# Autodesk Inventor assembly: dish_print
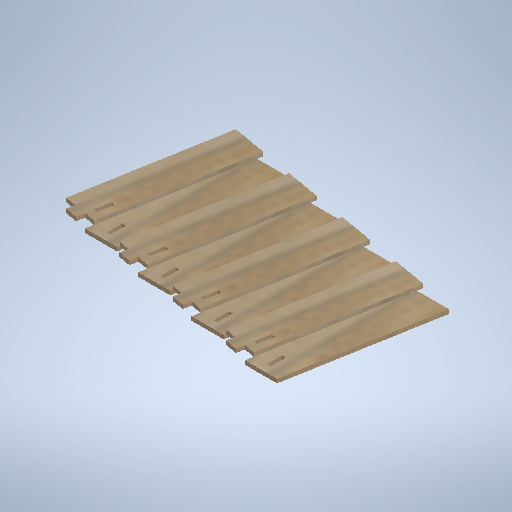
[picture p0: Inventor's stored thumbnail of the model, 512x512]
Saved by Autodesk Inventor 2026.1 (Build 301233020, 233B)
## iProperties
Created: 2025-10-27
Part Number: dish_print
Document SubType Name: Assembly
Designer: hibik
Author: hibik
## Documents named in this file (3)
- C:\Users\hibik\Documents\Robomech\conveyer\belt\dish_print.iam
- C:\Users\hibik\Documents\Robomech\conveyer\belt\dish_under.ipt
- C:\Users\hibik\Documents\Robomech\conveyer\belt\dish_upper.ipt
## Components (8 placed, 2 different names)
1. dish_under:1 — メイト:1, メイト:2, メイト:3
2. dish_upper:1 — メイト:1, メイト:2, メイト:3, フラッシュ:1, メイト:7, メイト:8
3. dish_under:2 — メイト:7, メイト:8
4. dish_upper:2 — フラッシュ:1, メイト:17, フラッシュ:3, メイト:18
5. dish_under:3 — メイト:17, メイト:18
6. dish_upper:3 — フラッシュ:3
7. dish_under:4
8. dish_upper:4
## Relationships (21: Mate 18, Flush 3)
- メイト:1 [Mate]: dish_under:1 ↔ dish_upper:1
- メイト:2 [Mate]: dish_under:1 ↔ dish_upper:1
- メイト:3 [Mate]: dish_under:1 ↔ dish_upper:1
- [Mate]: dish_under:2 ↔ dish_upper:2
- [Mate]: dish_under:2 ↔ dish_upper:2
- [Mate]: dish_under:2 ↔ dish_upper:2
- フラッシュ:1 [Flush]: dish_upper:1 ↔ dish_upper:2
- メイト:7 [Mate]: dish_upper:1 ↔ dish_under:2
- メイト:8 [Mate]: dish_upper:1 ↔ dish_under:2
- [Mate]: dish_under:3 ↔ dish_upper:3
- [Mate]: dish_under:3 ↔ dish_upper:3
- [Mate]: dish_under:3 ↔ dish_upper:3
- [Mate]: dish_under:4 ↔ dish_upper:4
- [Mate]: dish_under:4 ↔ dish_upper:4
- [Mate]: dish_under:4 ↔ dish_upper:4
- [Flush]: dish_upper:3 ↔ dish_upper:4
- [Mate]: dish_upper:3 ↔ dish_under:4
- [Mate]: dish_upper:3 ↔ dish_under:4
- メイト:17 [Mate]: dish_upper:2 ↔ dish_under:3
- フラッシュ:3 [Flush]: dish_upper:2 ↔ dish_upper:3
- メイト:18 [Mate]: dish_upper:2 ↔ dish_under:3
## Named parameters: d3_d0 = 0 mm, d4_d1 = 0 mm, d5_d2 = 0 mm, d9_d0 = 0 mm, d10_d1 = 0 mm, d11_d2 = 0 mm, d12_d3_d0 = 0 mm, d13_d4_d1 = 0 mm, d14_d5_d2 = 0 mm, d15_d6 = 0 mm, d16_d7 = 0 mm, d17_d8 = 0 mm
